# Autodesk Inventor assembly: Flywheel Design 2
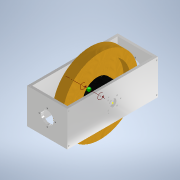
[picture p0: Inventor's stored thumbnail of the model, 180x180]
Saved by Autodesk Inventor 2020.2 (Build 242310000, 310)
## iProperties
Created: 2020-05-01
Part Number: Flywheel Design 2
Document SubType Name: Assembly
Designer: user
Author: user
## Documents named in this file (9)
- C:\Users\user\OneDrive\바탕 화면\Flywheel Design 2.iam
- C:\Users\user\OneDrive\바탕 화면\FWheel Side2.ipt
- C:\Users\user\OneDrive\바탕 화면\dd\FWheel Bottom.ipt
- C:\Users\user\OneDrive\바탕 화면\dd\FWheel Side.ipt
- C:\Users\user\OneDrive\바탕 화면\BARR608ZZ_Autodesk_Inventor_2020_20200501\AIS2020\BARR608ZZ.iam
- C:\Users\user\OneDrive\바탕 화면\dd\Stator.iam
- C:\Users\user\OneDrive\바탕 화면\dd\Rotor2.ipt
- C:\Users\user\OneDrive\바탕 화면\플라이~2\플라이휠+샤프트홀더.iam
- C:\Users\user\OneDrive\바탕 화면\Shaft.ipt
## Components (9 placed, 8 different names)
1. FWheel Side2:1 — Mate:10, Mate:11, Mate:12, Mate:22, Mate:23, Mate:24
2. FWheel Bottom:1 — Mate:1, Mate:2, Mate:3, Mate:23, Mate:24
3. FWheel Bottom:2 — Mate:4, Mate:5, Mate:6, Mate:22
4. FWheel Side:1 — Mate:1, Mate:2, Mate:3, Mate:4, Mate:5, Mate:6, Mate:13, Mate:14, Mate:15
5. BARR608ZZ:1 [sub-assembly] — Mate:10, Mate:11, Mate:12, Mate:20
6. Stator:1 [sub-assembly] — Mate:13, Mate:14, Mate:15, Mate:16, Flush:1, Mate:17
7. Rotor2:1 — Mate:16, Flush:1, Mate:18, Mate:19
8. 플라이휠+샤프트홀더:1 [sub-assembly] — Mate:17, Mate:18, Mate:19, Mate:21
9. Shaft:1 — Mate:20, Mate:21
## Relationships (22: Mate 21, Flush 1)
- Mate:1: FWheel Bottom:1 ↔ FWheel Side:1
- Mate:2: FWheel Bottom:1 ↔ FWheel Side:1
- Mate:3: FWheel Bottom:1 ↔ FWheel Side:1
- Mate:4: FWheel Bottom:2 ↔ FWheel Side:1
- Mate:5: FWheel Bottom:2 ↔ FWheel Side:1
- Mate:6: FWheel Bottom:2 ↔ FWheel Side:1
- Mate:10: FWheel Side2:1 ↔ BARR608ZZ:1
- Mate:11: FWheel Side2:1 ↔ BARR608ZZ:1
- Mate:12: FWheel Side2:1 ↔ BARR608ZZ:1
- Mate:13: FWheel Side:1 ↔ Stator:1
- Mate:14: FWheel Side:1 ↔ Stator:1
- Mate:15: FWheel Side:1 ↔ Stator:1
- Mate:16: Stator:1 ↔ Rotor2:1
- Flush:1 (6 mm): Stator:1 ↔ Rotor2:1
- Mate:17: Stator:1 ↔ 플라이휠+샤프트홀더:1
- Mate:18: Rotor2:1 ↔ 플라이휠+샤프트홀더:1
- Mate:19: Rotor2:1 ↔ 플라이휠+샤프트홀더:1
- Mate:20: BARR608ZZ:1 ↔ Shaft:1
- Mate:21: 플라이휠+샤프트홀더:1 ↔ Shaft:1
- Mate:22: FWheel Side2:1 ↔ FWheel Bottom:2
- Mate:23: FWheel Side2:1 ↔ FWheel Bottom:1
- Mate:24: FWheel Side2:1 ↔ FWheel Bottom:1
